# Autodesk Inventor assembly: Drive V3
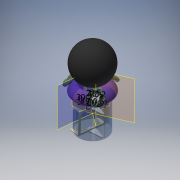
[picture p0: Inventor's stored thumbnail of the model, 180x180]
Saved by Autodesk Inventor 2019.1 (Build 231200000, 200)
## iProperties
Created: 2018-06-30
Part Number: Drive V3
Material: Generisch
Document SubType Name: Assembly
Designer: JochenAlt
Author: JochenAlt
## Documents named in this file (4)
- D:\Projects\Ondine\CAD\Drive V3.iam
- D:\Projects\Ondine\CAD\Sphere.ipt
- D:\Projects\Ondine\CAD\DriveChain V3.iam
- D:\Projects\Ondine\CAD\PCB\ControllerPCBHolder.ipt
## Components (5 placed, 3 different names)
1. Sphere:1 — Passend:38
2. DriveChain V3:1 [sub-assembly] — Passend:42, Passend:45, Passend:46, Passend:48
3. DriveChain V3:2 [sub-assembly] — Passend:42, Passend:47
4. DriveChain V3:3 [sub-assembly] — Passend:45, Passend:46, Passend:47
5. PCBHolder:1
## Relationships (6: Mate 6)
- Passend:38 [Mate]: Sphere:1
- Passend:42 [Mate]: DriveChain V3:1 ↔ DriveChain V3:2
- Passend:45 [Mate]: DriveChain V3:1 ↔ DriveChain V3:3
- Passend:46 [Mate]: DriveChain V3:1 ↔ DriveChain V3:3
- Passend:47 [Mate]: DriveChain V3:2 ↔ DriveChain V3:3
- Passend:48 [Mate]: DriveChain V3:1
